# Autodesk Inventor assembly: U assembly
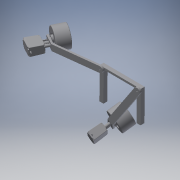
[picture p0: Inventor's stored thumbnail of the model, 180x180]
Saved by Autodesk Inventor 2019 (Build 230136000, 136)
## iProperties
Created: 2019-10-08
Part Number: U assembly
Document SubType Name: Assembly
Designer: Delta
Author: Delta
## Documents named in this file (6)
- C:\Robotics\CAD\2019-20_CAD\Collection\U assembly.iam
- C:\Robotics\CAD\2019-20_CAD\Collection\U-Part Gen 2.ipt
- C:\Robotics\CAD\2019-20_CAD\Collection\Wheel Arms.ipt
- C:\Robotics\CAD\COTSParts\Vex\2-Wire_Motor_393_276-2177.iam
- C:\Robotics\CAD\COTSParts\Wheels\2.5inFoamWheel250TMD.ipt
- C:\Robotics\CAD\2019-20_CAD\Collection\Shaft adapter 2.iam
## Components (9 placed, 5 different names)
1. U-Part Gen 2:1 — Mate:1, Mate:2, Mate:3, Mate:4
2. Wheel Arms:1 — Mate:1, Mate:2, Mate:31, Mate:32, Mate:33
3. Wheel Arms:2 — Mate:3, Mate:4, Mate:34, Mate:35, Mate:36
4. 2-Wire_Motor_393_276-2177:1 [sub-assembly] — Mate:34, Mate:35, Mate:36, Mate:46, Mate:47, Mate:48
5. 2-Wire_Motor_393_276-2177:2 [sub-assembly] — Mate:31, Mate:32, Mate:33, Mate:43, Mate:44, Mate:45
6. 2.5inFoamWheel250TMD:1 — Mate:40, Mate:41, Mate:42
7. 2.5inFoamWheel250TMD:2 — Mate:37, Mate:38, Mate:39
8. Shaft adapter 2:1 [sub-assembly] — Mate:40, Mate:41, Mate:42, Mate:43, Mate:44, Mate:45
9. Shaft adapter 2:2 [sub-assembly] — Mate:37, Mate:38, Mate:39, Mate:46, Mate:47, Mate:48
## Relationships (22: Mate 22)
- Mate:1: U-Part Gen 2:1 ↔ Wheel Arms:1
- Mate:2: U-Part Gen 2:1 ↔ Wheel Arms:1
- Mate:3: U-Part Gen 2:1 ↔ Wheel Arms:2
- Mate:4: U-Part Gen 2:1 ↔ Wheel Arms:2
- Mate:31: Wheel Arms:1 ↔ 2-Wire_Motor_393_276-2177:2
- Mate:32: Wheel Arms:1 ↔ 2-Wire_Motor_393_276-2177:2
- Mate:33: Wheel Arms:1 ↔ 2-Wire_Motor_393_276-2177:2
- Mate:34: Wheel Arms:2 ↔ 2-Wire_Motor_393_276-2177:1
- Mate:35: Wheel Arms:2 ↔ 2-Wire_Motor_393_276-2177:1
- Mate:36: Wheel Arms:2 ↔ 2-Wire_Motor_393_276-2177:1
- Mate:37: 2.5inFoamWheel250TMD:2 ↔ Shaft adapter 2:2
- Mate:38: 2.5inFoamWheel250TMD:2 ↔ Shaft adapter 2:2
- Mate:39: 2.5inFoamWheel250TMD:2 ↔ Shaft adapter 2:2
- Mate:40: 2.5inFoamWheel250TMD:1 ↔ Shaft adapter 2:1
- Mate:41: 2.5inFoamWheel250TMD:1 ↔ Shaft adapter 2:1
- Mate:42: 2.5inFoamWheel250TMD:1 ↔ Shaft adapter 2:1
- Mate:43: 2-Wire_Motor_393_276-2177:2 ↔ Shaft adapter 2:1
- Mate:44: 2-Wire_Motor_393_276-2177:2 ↔ Shaft adapter 2:1
- Mate:45: 2-Wire_Motor_393_276-2177:2 ↔ Shaft adapter 2:1
- Mate:46: 2-Wire_Motor_393_276-2177:1 ↔ Shaft adapter 2:2
- Mate:47: 2-Wire_Motor_393_276-2177:1 ↔ Shaft adapter 2:2
- Mate:48: 2-Wire_Motor_393_276-2177:1 ↔ Shaft adapter 2:2
